# Autodesk Inventor assembly: Camera_mount_01
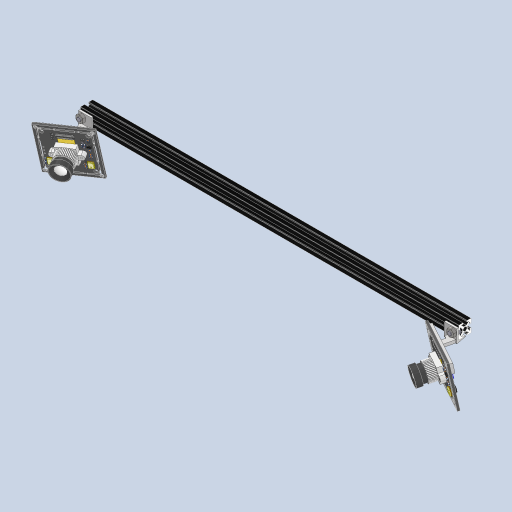
[picture p0: Inventor's stored thumbnail of the model, 512x512]
Saved by Autodesk Inventor 2024.4 (Build 284460000, 460)
## iProperties
Created: 2026-04-06
Part Number: Camera_mount_01
Document SubType Name: Assembly
Designer: tooles01
Author: tooles01
## Documents named in this file (4)
- C:\Users\tooles01\NYU Langone Health Dropbox\Shannon Toole\Shannon_Dropbox\Mar lab\RFID\camera_mount_angled\Camera_mount_01.iam
- C:\Users\tooles01\NYU Langone Health Dropbox\Shannon Toole\Shannon_Dropbox\Mar lab\Inventor_Lib\100078 MB BE BL 300mm.ipt
- C:\Users\tooles01\NYU Langone Health Dropbox\Shannon Toole\Shannon_Dropbox\Mar lab\RFID\camera_mount_angled\mount_04.iam
- C:\Users\tooles01\NYU Langone Health Dropbox\Shannon Toole\Shannon_Dropbox\Mar lab\RFID\camera_mount_angled\mount_04_mirror.iam
## Components (3 placed, 3 different names)
1. 100078 MB BE BL 300mm:1 — angle piece flush to post:1, M3 to post:1, M3 centered to post:1, angle piece flush to post end:1, angle piece to post bottom:1, angle piece flush to post:2, M3 to post:2, angle piece flush to post end:2, angle piece to post bottom:2
2. mount_04:1 [sub-assembly] — angle piece flush to post:1, M3 to post:1, M3 centered to post:1, angle piece flush to post end:1, angle piece to post bottom:1
3. mount_04_mirror:1 [sub-assembly] — angle piece flush to post:2, M3 to post:2, angle piece flush to post end:2, angle piece to post bottom:2
## Relationships (9: Mate 7, Flush 2)
- angle piece flush to post:1 [Mate]: 100078 MB BE BL 300mm:1 ↔ mount_04:1
- M3 to post:1 [Mate] (1 mm): 100078 MB BE BL 300mm:1 ↔ mount_04:1
- M3 centered to post:1 [Mate]: 100078 MB BE BL 300mm:1 ↔ mount_04:1
- angle piece flush to post end:1 [Flush]: 100078 MB BE BL 300mm:1 ↔ mount_04:1
- angle piece to post bottom:1 [Mate]: 100078 MB BE BL 300mm:1 ↔ mount_04:1
- angle piece flush to post:2 [Mate]: 100078 MB BE BL 300mm:1 ↔ mount_04_mirror:1
- M3 to post:2 [Mate] (1 mm): 100078 MB BE BL 300mm:1 ↔ mount_04_mirror:1
- angle piece flush to post end:2 [Flush]: 100078 MB BE BL 300mm:1 ↔ mount_04_mirror:1
- angle piece to post bottom:2 [Mate]: 100078 MB BE BL 300mm:1 ↔ mount_04_mirror:1
